# Autodesk Inventor assembly: Bridge
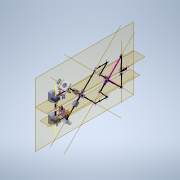
[picture p0: Inventor's stored thumbnail of the model, 180x180]
Saved by Autodesk Inventor 2020 (Build 240168000, 168)
## iProperties
Created: 2016-11-29
Part Number: Bridge
Document SubType Name: Assembly
Designer: map
Author: map
## Documents named in this file (20)
- C:\Users\whgu0532\Documents\4Pi\4Pi-Oxford\01-Bridge.iam
- C:\Users\whgu0532\Documents\4Pi\4Pi-Oxford\__MASTER__.ipt
- C:\Users\whgu0532\Documents\4Pi\4Pi-Oxford\FAB-P0018 - Mirror Mount - U100.ipt
- C:\Users\whgu0532\Documents\4Pi\4Pi-Oxford\FAB-P0028 - Lens Mount, LMR1.ipt
- C:\Users\whgu0532\Documents\4Pi\4Pi-Oxford\FAB-P0029- Filter Cube Support-Upper.ipt
- C:\Users\whgu0532\Documents\4Pi\4Pi-Oxford\FAB-P0032 - Filter Cube Excitation V2.ipt
- C:\Users\whgu0532\Documents\4Pi\4Pi-Oxford\FAB-P0033- Filter Cube- Emission.ipt
- C:\Users\whgu0532\Documents\4Pi\4Pi-Oxford\PRM05_3.ipt
- C:\Users\whgu0532\Documents\4Pi\4Pi-Oxford\SS100-F3H.ipt
- C:\Users\whgu0532\Documents\4Pi\4Pi-Oxford\Thor LMR1-M Fixed Lens Mt.ipt
- C:\Users\whgu0532\Documents\4Pi\4Pi-Oxford\U100-A3H.ipt
- C:\Users\whgu0532\Documents\4Pi\4Pi-Oxford\__CAVITY_AND_IMAGING_OPTICS__.iam
- C:\Users\whgu0532\Documents\4Pi\4Pi-Oxford\FAB-P0027 - Mirror Mount, 45 deg - U100.ipt
- C:\Users\whgu0532\Documents\4Pi\4Pi-Oxford\Thor ST1XY-A-M.ipt
- C:\Users\whgu0532\Documents\4Pi\4Pi-Oxford\LP-2A mount.ipt
- C:\Users\whgu0532\Documents\4Pi\4Pi-Oxford\LP-2A update.ipt
- C:\Users\whgu0532\Documents\4Pi\4Pi-Oxford\BostonDM.iam
- C:\Users\whgu0532\Documents\4Pi\4Pi-Oxford\U100-A-LH-3H.ipt
- C:\Users\whgu0532\Documents\4Pi\4Pi-Oxford\FAB-OX0016-FilterCubeSupport.Lower.Derived.ipt
- C:\Users\whgu0532\Documents\4Pi\R2017\en-US\ISO 4762(1)\DIN EN ISO 4762 - M4 x 20.ipt
## Components (36 placed, 19 different names)
1. __MASTER__:1 — Angle:3, Mate:65, Mate:66, Mate:69, Mate:90, Mate:91
2. __CAVITY_AND_IMAGING_OPTICS__:1 [sub-assembly] — Mate:1, Mate:2, Mate:3, Tangent:1, Mate:15, Mate:16, Mate:26, Tangent:2, Mate:34, Mate:54, Mate:55, Mate:61, Mate:67, Mate:68, Mate:80, Mate:82, Flush:7, Flush:8, Mate:84, Mate:85
3. FAB-OX0016-FilterCubeSupport.Lower.Derived:1 — Mate:51, Mate:52, Mate:56, Mate:59, Mate:60, Angle:5, Angle:7, Mate:70
4. PRM05_3:1 — Mate:43, Mate:44, Mate:65
5. SS100-F3H:1 — Mate:13, Mate:14, Mate:72, Mate:88, Mate:92
6. Thor LMR1-M Fixed Lens Mt:1 — Mate:1, Mate:7, Mate:8, Tangent:1
7. U100-A3H:1 — Mate:2, Mate:3, Mate:4, Angle:13, Mate:86
8. FAB-P0029- FilterCubeSupport.Upper:1 — Mate:17, Mate:33, Mate:35, Mate:42, Mate:43, Mate:44, Mate:47, Angle:6, Mate:96
9. FAB-P0028 - Lens Mount, LMR1:1 — Mate:7, Mate:8, Mate:9
10. FAB-P0018 - Mirror Mount - U100:1 — Mate:4, Mate:10, Angle:13, Mate:86, Symmetry:1, Symmetry:2
11. FAB-P0027 - Mirror Mount, 45 deg - U100:1 — Mate:11, Mate:13, Mate:14, Mate:32, Flush:2, Angle:3, Mate:88, Symmetry:3
12. SS100-F3H:2 — Mate:15, Mate:16, Mate:17
13. FAB-P0018 - Mirror Mount - U100:2 — Mate:25, Angle:12, Mate:81, Angle:14, Mate:87, Symmetry:1, Symmetry:2
14. U100-A-LH-3H:1 — Mate:80, Angle:12, Mate:81, Mate:82, Angle:14, Mate:87
15. FAB-P0028 - Lens Mount, LMR1:2 — Mate:27
16. Thor LMR1-M Fixed Lens Mt:2 — Mate:26, Tangent:2
17. SS100-F3H:3 — Mate:29, Mate:71, Mate:89
18. FAB-P0027 - Mirror Mount, 45 deg - U100:2 — Mate:29, Mate:31, Flush:2, Mate:89, Symmetry:3
19. Thor ST1XY-A-M:1 — Mate:33, Mate:34, Mate:35
20. FAB-P0032 - Filter Cube Excitation V2:1 — Mate:37, Mate:39, Mate:42, Mate:46, Mate:66, Mate:96
21. FAB-P0033- Filter Cube- Emission:1 — Mate:37, Mate:39, Mate:46, Insert:3, Insert:4
22. FAB-P0032 - Filter Cube Excitation V2:2 — Mate:48, Mate:49, Mate:68, Mate:69, Mate:70
23. FAB-P0033- Filter Cube- Emission:2 — Mate:48, Mate:49, Insert:1, Insert:2
24. PRM05_3:2 — Mate:56, Mate:67
25. SS100-F3H:4 — Mate:52, Mate:54, Mate:55
26. Thor ST1XY-A-M:2 — Mate:59, Mate:60, Mate:61
27. LP-2A mount:1 — Angle:10, Mate:93
28. BostonDM:1 [sub-assembly] — Flush:8, Mate:84
29. LP-2A update:1 — Mate:93
30. BostonDM:2 [sub-assembly] — Flush:7, Mate:85
31. LP-2A update:2 — Angle:11, Mate:94, Flush:9, Mate:95
32. LP-2A mount:2 — Mate:94, Flush:9, Mate:95
33. DIN EN ISO 4762 M4 x 20:1 — Insert:1
34. DIN EN ISO 4762 M4 x 20:2 — Insert:2
35. DIN EN ISO 4762 M4 x 20:3 — Insert:3
36. DIN EN ISO 4762 M4 x 20:4 — Insert:4
## Relationships (99: Mate 71, Angle 11, Flush 8, Insert 4, Symmetry 3, Tangent 2)
- Mate:1: __CAVITY_AND_IMAGING_OPTICS__:1 ↔ Thor LMR1-M Fixed Lens Mt:1
- Mate:2: __CAVITY_AND_IMAGING_OPTICS__:1 ↔ U100-A3H:1
- Mate:3: __CAVITY_AND_IMAGING_OPTICS__:1 ↔ U100-A3H:1
- Mate:4: U100-A3H:1 ↔ FAB-P0018 - Mirror Mount - U100:1
- Mate:7: Thor LMR1-M Fixed Lens Mt:1 ↔ FAB-P0028 - Lens Mount, LMR1:1
- Mate:8: Thor LMR1-M Fixed Lens Mt:1 ↔ FAB-P0028 - Lens Mount, LMR1:1
- Tangent:1 (-1.275 mm): __CAVITY_AND_IMAGING_OPTICS__:1 ↔ Thor LMR1-M Fixed Lens Mt:1
- Flush:1 (-70 mm)
- Mate:9: FAB-P0028 - Lens Mount, LMR1:1
- Mate:10: FAB-P0018 - Mirror Mount - U100:1
- Mate:11: FAB-P0027 - Mirror Mount, 45 deg - U100:1
- Mate:13: SS100-F3H:1 ↔ FAB-P0027 - Mirror Mount, 45 deg - U100:1
- Mate:14: SS100-F3H:1 ↔ FAB-P0027 - Mirror Mount, 45 deg - U100:1
- Mate:15: __CAVITY_AND_IMAGING_OPTICS__:1 ↔ SS100-F3H:2
- Mate:16: __CAVITY_AND_IMAGING_OPTICS__:1 ↔ SS100-F3H:2
- Mate:17: FAB-P0029- FilterCubeSupport.Upper:1 ↔ SS100-F3H:2
- [Mate]: FAB-P0028 - Lens Mount, LMR1:2 ↔ Thor LMR1-M Fixed Lens Mt:2
- [Mate]: FAB-P0028 - Lens Mount, LMR1:2 ↔ Thor LMR1-M Fixed Lens Mt:2
- Mate:25: FAB-P0018 - Mirror Mount - U100:2
- Mate:26: __CAVITY_AND_IMAGING_OPTICS__:1 ↔ Thor LMR1-M Fixed Lens Mt:2
- Tangent:2 (-1.275 mm): __CAVITY_AND_IMAGING_OPTICS__:1 ↔ Thor LMR1-M Fixed Lens Mt:2
- Mate:27: FAB-P0028 - Lens Mount, LMR1:2
- Mate:29: SS100-F3H:3 ↔ FAB-P0027 - Mirror Mount, 45 deg - U100:2
- [Mate]: SS100-F3H:3 ↔ FAB-P0027 - Mirror Mount, 45 deg - U100:2
- Mate:31: FAB-P0027 - Mirror Mount, 45 deg - U100:2
- Mate:32: FAB-P0027 - Mirror Mount, 45 deg - U100:1
- Flush:2: FAB-P0027 - Mirror Mount, 45 deg - U100:1 ↔ FAB-P0027 - Mirror Mount, 45 deg - U100:2
- Angle:3 (180 deg): __MASTER__:1 ↔ FAB-P0027 - Mirror Mount, 45 deg - U100:1
- Mate:33: FAB-P0029- FilterCubeSupport.Upper:1 ↔ Thor ST1XY-A-M:1
- Mate:34: __CAVITY_AND_IMAGING_OPTICS__:1 ↔ Thor ST1XY-A-M:1
- Mate:35: FAB-P0029- FilterCubeSupport.Upper:1 ↔ Thor ST1XY-A-M:1
- Mate:37: FAB-P0032 - Filter Cube Excitation V2:1 ↔ FAB-P0033- Filter Cube- Emission:1
- Mate:39: FAB-P0032 - Filter Cube Excitation V2:1 ↔ FAB-P0033- Filter Cube- Emission:1
- Mate:42: FAB-P0029- FilterCubeSupport.Upper:1 ↔ FAB-P0032 - Filter Cube Excitation V2:1
- Mate:43: PRM05_3:1 ↔ FAB-P0029- FilterCubeSupport.Upper:1
- Mate:44: PRM05_3:1 ↔ FAB-P0029- FilterCubeSupport.Upper:1
- Mate:46: FAB-P0032 - Filter Cube Excitation V2:1 ↔ FAB-P0033- Filter Cube- Emission:1
- Mate:47: FAB-P0029- FilterCubeSupport.Upper:1
- Mate:48: FAB-P0032 - Filter Cube Excitation V2:2 ↔ FAB-P0033- Filter Cube- Emission:2
- Mate:49: FAB-P0032 - Filter Cube Excitation V2:2 ↔ FAB-P0033- Filter Cube- Emission:2
- [Mate]: FAB-P0032 - Filter Cube Excitation V2:2 ↔ FAB-P0033- Filter Cube- Emission:2
- Mate:51: FAB-OX0016-FilterCubeSupport.Lower.Derived:1
- Mate:54: __CAVITY_AND_IMAGING_OPTICS__:1 ↔ SS100-F3H:4
- Mate:55: __CAVITY_AND_IMAGING_OPTICS__:1 ↔ SS100-F3H:4
- Mate:61: __CAVITY_AND_IMAGING_OPTICS__:1 ↔ Thor ST1XY-A-M:2
- Angle:6 (0 deg): FAB-P0029- FilterCubeSupport.Upper:1
- Mate:65: __MASTER__:1 ↔ PRM05_3:1
- Mate:66: __MASTER__:1 ↔ FAB-P0032 - Filter Cube Excitation V2:1
- Mate:67: __CAVITY_AND_IMAGING_OPTICS__:1 ↔ PRM05_3:2
- Mate:68: __CAVITY_AND_IMAGING_OPTICS__:1 ↔ FAB-P0032 - Filter Cube Excitation V2:2
- Mate:69: __MASTER__:1 ↔ FAB-P0032 - Filter Cube Excitation V2:2
- Angle:8 (0 deg)
- Mate:71: SS100-F3H:3
- Angle:9 (0 deg)
- Mate:72: SS100-F3H:1
- Angle:10 (0 deg): LP-2A mount:1
- [Flush]: LP-2A mount:1 ↔ LP-2A update:1
- [Mate]: LP-2A mount:1 ↔ LP-2A update:1
- [Mate]: BostonDM:1 ↔ LP-2A update:1
- [Flush] (0.005 mm): BostonDM:1 ↔ LP-2A update:1
- [Mate]: BostonDM:2 ↔ LP-2A update:2
- [Flush] (0.005 mm): BostonDM:2 ↔ LP-2A update:2
- Angle:11 (180 deg): LP-2A update:2
- Mate:80: __CAVITY_AND_IMAGING_OPTICS__:1 ↔ U100-A-LH-3H:1
- Angle:12 (0 deg): FAB-P0018 - Mirror Mount - U100:2 ↔ U100-A-LH-3H:1
- Mate:81: FAB-P0018 - Mirror Mount - U100:2 ↔ U100-A-LH-3H:1
- Mate:82: __CAVITY_AND_IMAGING_OPTICS__:1 ↔ U100-A-LH-3H:1
- Flush:7: __CAVITY_AND_IMAGING_OPTICS__:1 ↔ BostonDM:2
- Flush:8: __CAVITY_AND_IMAGING_OPTICS__:1 ↔ BostonDM:1
- Mate:84: __CAVITY_AND_IMAGING_OPTICS__:1 ↔ BostonDM:1
- Mate:85: __CAVITY_AND_IMAGING_OPTICS__:1 ↔ BostonDM:2
- Angle:13 (0 deg): U100-A3H:1 ↔ FAB-P0018 - Mirror Mount - U100:1
- Mate:86: U100-A3H:1 ↔ FAB-P0018 - Mirror Mount - U100:1
- Angle:14 (0 deg): FAB-P0018 - Mirror Mount - U100:2 ↔ U100-A-LH-3H:1
- Mate:87 (60.77 mm): FAB-P0018 - Mirror Mount - U100:2 ↔ U100-A-LH-3H:1
- Mate:88: SS100-F3H:1 ↔ FAB-P0027 - Mirror Mount, 45 deg - U100:1
- Mate:89: SS100-F3H:3 ↔ FAB-P0027 - Mirror Mount, 45 deg - U100:2
- Mate:90: __MASTER__:1
- Mate:91: __MASTER__:1
- Mate:92 (-91 mm): SS100-F3H:1
- Mate:93: LP-2A mount:1 ↔ LP-2A update:1
- Mate:94: LP-2A update:2 ↔ LP-2A mount:2
- Flush:9: LP-2A update:2 ↔ LP-2A mount:2
- Mate:95: LP-2A update:2 ↔ LP-2A mount:2
- Symmetry:1: FAB-P0018 - Mirror Mount - U100:1 ↔ FAB-P0018 - Mirror Mount - U100:2
- Symmetry:2: FAB-P0018 - Mirror Mount - U100:1 ↔ FAB-P0018 - Mirror Mount - U100:2
- Symmetry:3: FAB-P0027 - Mirror Mount, 45 deg - U100:1 ↔ FAB-P0027 - Mirror Mount, 45 deg - U100:2
- Mate:96: FAB-P0029- FilterCubeSupport.Upper:1 ↔ FAB-P0032 - Filter Cube Excitation V2:1
- Mate:52: FAB-OX0016-FilterCubeSupport.Lower.Derived:1 ↔ SS100-F3H:4
- Mate:56: FAB-OX0016-FilterCubeSupport.Lower.Derived:1 ↔ PRM05_3:2
- Mate:59: FAB-OX0016-FilterCubeSupport.Lower.Derived:1 ↔ Thor ST1XY-A-M:2
- Mate:60: FAB-OX0016-FilterCubeSupport.Lower.Derived:1 ↔ Thor ST1XY-A-M:2
- Angle:5 (0 deg): FAB-OX0016-FilterCubeSupport.Lower.Derived:1
- Angle:7 (0 deg): FAB-OX0016-FilterCubeSupport.Lower.Derived:1
- Mate:70: FAB-OX0016-FilterCubeSupport.Lower.Derived:1 ↔ FAB-P0032 - Filter Cube Excitation V2:2
- Insert:1: FAB-P0033- Filter Cube- Emission:2 ↔ DIN EN ISO 4762 M4 x 20:1
- Insert:2: FAB-P0033- Filter Cube- Emission:2 ↔ DIN EN ISO 4762 M4 x 20:2
- Insert:3: FAB-P0033- Filter Cube- Emission:1 ↔ DIN EN ISO 4762 M4 x 20:3
- Insert:4: FAB-P0033- Filter Cube- Emission:1 ↔ DIN EN ISO 4762 M4 x 20:4
## Named parameters: d36_d11 = 0 mm, d37_d12 = 0 mm, d47_d21 = 0 mm, d48_d22 = 0 mm, d74_d62 = 0 mm, d75_d72 = 0 mm, d76_d60 = 0 mm, d127_d2 = 0 mm, d130_d5 = 0.005 mm, d133_d127_d2 = 0 mm, d134_d130_d5 = 0.005 mm
